# Autodesk Inventor assembly: human 01
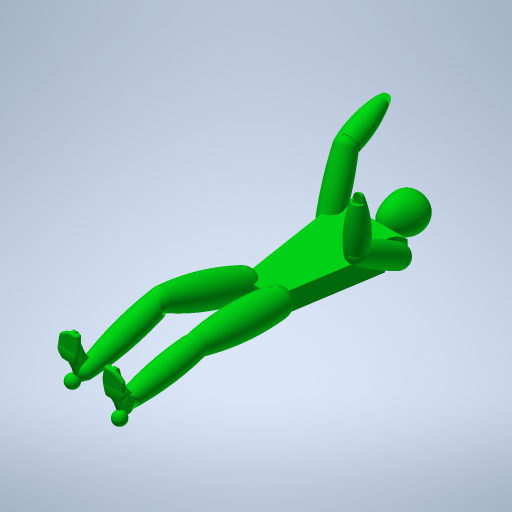
[picture p0: Inventor's stored thumbnail of the model, 512x512]
Saved by Autodesk Inventor 2023.1 (Build 271208000, 208)
## iProperties
Created: 2018-05-21
Part Number: human 01
Material: Типовые
Document SubType Name: Assembly
Designer: admin
Stock Number: Dummy
Author: admin
## Documents named in this file (14)
- H:\Other computers\My Computer\Inventor\Nadyim\CAD\32degree straight\CAD\dummi\human 01\human 01.iam
- H:\Other computers\My Computer\Inventor\Nadyim\CAD\32degree straight\CAD\dummi\human 01\Dimensions_sketch.ipt
- H:\Other computers\My Computer\Inventor\Nadyim\CAD\32degree straight\CAD\dummi\human 01\shoulder joint.ipt
- H:\Other computers\My Computer\Inventor\Nadyim\CAD\32degree straight\CAD\dummi\human 01\Shoulder parametric.ipt
- H:\Other computers\My Computer\Inventor\Nadyim\CAD\32degree straight\CAD\dummi\human 01\body parametric.ipt
- H:\Other computers\My Computer\Inventor\Nadyim\CAD\32degree straight\CAD\dummi\human 01\shoe parametric.ipt
- H:\Other computers\My Computer\Inventor\Nadyim\CAD\32degree straight\CAD\dummi\human 01\feet parametric.ipt
- H:\Other computers\My Computer\Inventor\Nadyim\CAD\32degree straight\CAD\dummi\human 01\Forearm.ipt
- H:\Other computers\My Computer\Inventor\Nadyim\CAD\32degree straight\CAD\dummi\human 01\Elbow.ipt
- H:\Other computers\My Computer\Inventor\Nadyim\CAD\32degree straight\CAD\dummi\human 01\Hip.ipt
- H:\Other computers\My Computer\Inventor\Nadyim\CAD\32degree straight\CAD\dummi\human 01\upper leg.ipt
- H:\Other computers\My Computer\Inventor\Nadyim\CAD\32degree straight\CAD\dummi\human 01\shank.ipt
- H:\Other computers\My Computer\Inventor\Nadyim\CAD\32degree straight\CAD\dummi\human 01\feet parametric_MIR.ipt
- H:\Other computers\My Computer\Inventor\Nadyim\CAD\32degree straight\CAD\dummi\human 01\Head.ipt
## Components (20 placed, 13 different names)
1. Dimensions_sketch:1
2. shoulder joint:1 — С поворотом:1, С поворотом:9
3. Shoulder parametric:1 — С поворотом:1, С поворотом:3
4. body parametric:1 — Заподлицо:2, С поворотом:9, Заподлицо:7, Заподлицо:8, С поворотом:10, С поворотом:14, С поворотом:15, Совмещение:1, Заподлицо:10
5. shoe parametric:1 — Заподлицо:3
6. feet parametric:1 — С поворотом:20
7. Forearm:1 — С поворотом:2
8. Elbow:1 — С поворотом:2, С поворотом:3
9. Hip:1 — С поворотом:14, С поворотом:19
10. upper leg:1 — С поворотом:19, С поворотом:17
11. upper leg:2 — С поворотом:18, С поворотом:16
12. Hip:2 — С поворотом:15, С поворотом:18
13. shank:1 — С поворотом:16, С поворотом:20
14. shank:2 — С поворотом:17, С поворотом:21
15. shoulder joint:2 — С поворотом:10, С поворотом:11
16. Shoulder parametric:2 — С поворотом:11, С поворотом:13
17. Elbow:2 — С поворотом:12, С поворотом:13
18. Forearm:2 — С поворотом:12
19. feet parametric_MIR:1 — С поворотом:21
20. Head:1 — Заподлицо:9, Совмещение:1, Заподлицо:10
## Relationships (23: RevoluteJoint 16, Flush 6, Mate 1)
- С поворотом:1 [RevoluteJoint]: shoulder joint:1 ↔ Shoulder parametric:1
- Заподлицо:2 [Flush]: body parametric:1
- Заподлицо:3 [Flush]: shoe parametric:1
- С поворотом:2 [RevoluteJoint]: Forearm:1 ↔ Elbow:1
- С поворотом:3 [RevoluteJoint]: Shoulder parametric:1 ↔ Elbow:1
- С поворотом:9 [RevoluteJoint]: shoulder joint:1 ↔ body parametric:1
- Заподлицо:7 [Flush]: body parametric:1
- Заподлицо:8 [Flush]: body parametric:1
- С поворотом:10 [RevoluteJoint]: body parametric:1 ↔ shoulder joint:2
- С поворотом:11 [RevoluteJoint]: shoulder joint:2 ↔ Shoulder parametric:2
- С поворотом:12 [RevoluteJoint]: Elbow:2 ↔ Forearm:2
- С поворотом:13 [RevoluteJoint]: Shoulder parametric:2 ↔ Elbow:2
- С поворотом:14 [RevoluteJoint]: body parametric:1 ↔ Hip:1
- С поворотом:15 [RevoluteJoint]: body parametric:1 ↔ Hip:2
- С поворотом:19 [RevoluteJoint]: Hip:1 ↔ upper leg:1
- С поворотом:18 [RevoluteJoint]: upper leg:2 ↔ Hip:2
- С поворотом:16 [RevoluteJoint]: upper leg:2 ↔ shank:1
- С поворотом:17 [RevoluteJoint]: upper leg:1 ↔ shank:2
- С поворотом:20 [RevoluteJoint]: feet parametric:1 ↔ shank:1
- С поворотом:21 [RevoluteJoint]: shank:2 ↔ feet parametric_MIR:1
- Заподлицо:9 [Flush]: Head:1
- Совмещение:1 [Mate] (100 mm): body parametric:1 ↔ Head:1
- Заподлицо:10 [Flush]: body parametric:1 ↔ Head:1
